# Autodesk Inventor assembly: 胴体_1
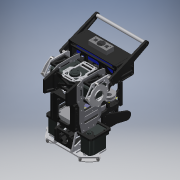
[picture p0: Inventor's stored thumbnail of the model, 180x180]
Saved by Autodesk Inventor 2018 (Build 220112000, 112)
## iProperties
Created: 2016-05-03
Part Number: 胴体_1
Document SubType Name: Assembly
Designer: hiroaki
Mass: 1394.39 g
Surface Area: 4542.63 cm^2
Volume: 847.153 cm^3
Density: 1.64598 g/cm^3
Author: hiroaki
## Documents named in this file (26)
- C:\Users\taka\Documents\github\OpenPlatform\mechanism\OpenPlatform_ver3_0\上半身\胴体\胴体_1.iam
- C:\Users\taka\Documents\github\OpenPlatform\mechanism\OpenPlatform_ver3_0\既製品\B3M11xx.ipt
- C:\Users\taka\Documents\github\OpenPlatform\mechanism\OpenPlatform_ver3_0\既製品\B3M10xx.ipt
- C:\Users\taka\Documents\github\OpenPlatform\mechanism\OpenPlatform_ver3_0\上半身\胴体\胴体_メインフレーム_1_1.ipt
- C:\Users\taka\Documents\github\OpenPlatform\mechanism\OpenPlatform_ver3_0\下半身\付け根ロール\付け根ロール_サブフレーム_1_3.ipt
- C:\Users\taka\Documents\github\OpenPlatform\mechanism\OpenPlatform_ver3_0\上半身\胴体\胴体_メインフレーム_1_2.ipt
- C:\Users\taka\Documents\github\OpenPlatform\mechanism\OpenPlatform_ver3_0\上半身\胴体\胴体_サブフレーム_1_1.ipt
- C:\Users\taka\Documents\github\OpenPlatform\mechanism\OpenPlatform_ver3_0\上半身\胴体\胴体_サブフレーム_1_2.ipt
- C:\Users\taka\Documents\github\OpenPlatform\mechanism\OpenPlatform_ver3_0\上半身\胴体\胴体_サブフレーム_1_3.ipt
- C:\Users\taka\Documents\github\OpenPlatform\mechanism\OpenPlatform_ver3_0\上半身\胴体\胴体_サブフレーム_1_4.ipt
- C:\Users\taka\Documents\github\OpenPlatform\mechanism\OpenPlatform_ver3_0\上半身\胴体\胴体_サブフレーム_1_6.ipt
- C:\Users\taka\Documents\github\OpenPlatform\mechanism\OpenPlatform_ver3_0\上半身\胴体\胴体_サブフレーム_1_6_MIR.ipt
- C:\Users\taka\Documents\github\OpenPlatform\mechanism\OpenPlatform_ver3_0\上半身\胴体\胴体_サブフレーム_1_1_MIR.ipt
- C:\Users\taka\Documents\github\OpenPlatform\mechanism\OpenPlatform_ver3_0\上半身\胴体\胴体_サブフレーム_1_7.ipt
- C:\Users\taka\Documents\github\OpenPlatform\mechanism\OpenPlatform_ver3_0\上半身\胴体\胴体_サブフレーム_1_7_MIR.ipt
- C:\Users\taka\Documents\github\OpenPlatform\mechanism\OpenPlatform_ver3_0\上半身\胴体\胴体_サブフレーム_1_9.ipt
- C:\Users\taka\Documents\github\OpenPlatform\mechanism\OpenPlatform_ver3_0\上半身\胴体\胴体_メインフレーム_1_12.ipt
- C:\Users\taka\Documents\github\OpenPlatform\mechanism\OpenPlatform_ver3_0\上半身\胴体\胴体_メインフレーム_1_13.ipt
- C:\Users\taka\Documents\github\OpenPlatform\mechanism\OpenPlatform_ver3_0\上半身\胴体\胴体_サブフレーム_1_10.ipt
- C:\Users\taka\Documents\github\OpenPlatform\mechanism\OpenPlatform_ver3_0\上半身\胴体\胴体_サブフレーム_1_11.ipt
- C:\Users\taka\Documents\github\OpenPlatform\mechanism\OpenPlatform_ver3_0\既製品\SLCG5_5-6.ipt
- C:\Users\taka\Documents\github\OpenPlatform\mechanism\OpenPlatform_ver3_0\既製品\ALSFB6-66.ipt
- C:\Users\taka\Documents\github\OpenPlatform\mechanism\OpenPlatform_ver3_0\上半身\コックピット\コックピット_2\コックピット_2.iam
- C:\Users\taka\Documents\github\OpenPlatform\mechanism\OpenPlatform_ver3_0\上半身\胴体\胴体_サブフレーム_1_12.ipt
- C:\Users\taka\Documents\github\OpenPlatform\mechanism\OpenPlatform_ver3_0\既製品\AETTF8-135-M3-N3.ipt
- C:\Users\taka\Documents\github\OpenPlatform\mechanism\OpenPlatform_ver3_0\既製品\SLCG5_5-8.ipt
## Components (60 placed, 24 different names)
1. 胴体_メインフレーム_1_1:1 — 挿入:1, 挿入:2, 挿入:3, 挿入:4, 挿入:5, 挿入:6, 挿入:43, 挿入:44, 挿入:120, 挿入:121, 挿入:194, 挿入:195, 挿入:196, 挿入:197, 挿入:198, 挿入:199, 挿入:200, 挿入:201, 角度:44
2. 付け根ロール_サブフレーム_1_3:1 — 挿入:218, 挿入:219, 挿入:220, 挿入:221
3. 胴体_メインフレーム_1_2:1 — 挿入:23, 挿入:24, 挿入:25, 挿入:28
4. 胴体_メインフレーム_1_12:1 — 挿入:148, 挿入:149, 挿入:150, 挿入:151
5. 胴体_サブフレーム_1_1:1 — 挿入:43, 挿入:44, 挿入:118, 挿入:119, メイト:9, メイト:10, メイト:11
6. 胴体_サブフレーム_1_2:1 — フラッシュ:1, メイト:3, メイト:4
7. 胴体_サブフレーム_1_3:1 — 挿入:150, 挿入:151, 挿入:162, 挿入:163, 挿入:168, 挿入:169, 挿入:192, 挿入:193, 挿入:228, 挿入:229, メイト:4, 挿入:231, 挿入:232, 挿入:236
8. 胴体_サブフレーム_1_4:1 — 挿入:57, 挿入:58, 挿入:148, 挿入:149, 挿入:152, 挿入:153, 挿入:206, 挿入:207, 挿入:208, 挿入:209, 挿入:248, 挿入:249
9. 胴体_サブフレーム_1_6:1 — 挿入:118, 挿入:119
10. 胴体_サブフレーム_1_7:1 — 挿入:231, 挿入:232
11. 胴体_サブフレーム_1_9:1 — 挿入:133, 挿入:134, 挿入:135
12. 胴体_サブフレーム_1_10:1 — 挿入:173, 挿入:174, 挿入:175, 挿入:176, 挿入:179, 挿入:188, 挿入:189
13. 胴体_サブフレーム_1_11:1 — 挿入:182, 挿入:183, 挿入:184, 挿入:185, 挿入:186, 挿入:187
14. 胴体_サブフレーム_1_12:1 — 挿入:247, 角度:35, 角度:36, 挿入:250, 挿入:251
15. 胴体_メインフレーム_1_13:1 — 挿入:188, 挿入:189, 挿入:190, 挿入:191, 挿入:192, 挿入:193
16. B3M11xx:5 — 挿入:175, 挿入:176, 挿入:179, 挿入:182, 挿入:183, 挿入:185, 挿入:186
17. B3M11xx:4 — 挿入:57, 挿入:58, 挿入:133, 挿入:134, 挿入:135, 角度:31, 角度:39
18. B3M11xx:3 — 角度:1, 挿入:76, 挿入:77, 挿入:130, 挿入:131, 挿入:132
19. B3M11xx:2 — 挿入:2, 挿入:4, 挿入:5, 挿入:23, 挿入:25, 角度:23, 角度:43
20. B3M11xx:1 — 角度:1, 挿入:1, 挿入:3, 挿入:6, 挿入:24, 挿入:28
21. SLCG5_5-6:1 — 挿入:200, 挿入:218, 角度:27, 角度:29
22. SLCG5_5-6:2 — 挿入:196, 挿入:222, 角度:25, 角度:28, 角度:43
23. SLCG5_5-6:3 — 挿入:198, 挿入:220, 角度:29
24. SLCG5_5-6:4 — 挿入:199, 挿入:219, 角度:30
25. SLCG5_5-6:5 — 挿入:204, 挿入:217, 角度:34
26. SLCG5_5-6:6 — 挿入:202, 挿入:216, 角度:42
27. SLCG5_5-6:7 — 挿入:197, 挿入:225, 角度:26
28. SLCG5_5-6:8 — 挿入:201, 挿入:221, 角度:28, 角度:30
29. SLCG5_5-6:9 — 挿入:206, 挿入:212, 角度:40
30. SLCG5_5-6:10 — 挿入:205, 挿入:215, 角度:41
31. SLCG5_5-6:11 — 挿入:203, 挿入:214, 角度:33, 角度:34
32. SLCG5_5-6:12 — 挿入:195, 挿入:224, 角度:25
33. SLCG5_5-6:13 — 挿入:207, 挿入:213, 角度:32
34. SLCG5_5-6:14 — 挿入:208, 挿入:211, 角度:31, 角度:32, 角度:33
35. SLCG5_5-6:15 — 挿入:209, 挿入:210, 角度:39, 角度:40, 角度:41, 角度:42
36. SLCG5_5-6:16 — 挿入:194, 挿入:223, 角度:23, 角度:26, 角度:27
37. ALSFB6-66:1 — 挿入:229, 挿入:230, メイト:3, メイト:9
38. ALSFB6-66:2 — 挿入:227, 挿入:228, メイト:1, メイト:2
39. ALSFB6-66:3 — メイト:10, メイト:11, 挿入:235, 挿入:236
40. コックピット_2:1 [sub-assembly] — 角度:44, メイト:14, メイト:15
41. AETTF8-135-M3-N3:1 — 挿入:246, 挿入:247
42. SLCG5_5-8:1 — 角度:38, 挿入:252, メイト:12
43. SLCG5_5-8:2 — 挿入:249, 角度:35, 挿入:251
44. SLCG5_5-8:3 — 角度:37, 挿入:253, メイト:13
45. SLCG5_5-8:4 — 挿入:248, 角度:36, 挿入:250
46. 胴体_サブフレーム_1_12:2 — 挿入:246, 角度:37, 角度:38, 挿入:252, 挿入:253
47. 胴体_メインフレーム_1_13:2 — 挿入:168, 挿入:169, 挿入:170, 挿入:171, 挿入:173, 挿入:174, 挿入:184, 挿入:187
48. 胴体_メインフレーム_1_12:2 — 挿入:152, 挿入:153, 挿入:162, 挿入:163
49. 胴体_メインフレーム_1_12:3 — 挿入:154, 挿入:155, 挿入:156, 挿入:157
50. 胴体_メインフレーム_1_12:4 — 挿入:158, 挿入:159, 挿入:160, 挿入:161
51. 胴体_サブフレーム_1_9:2 — 挿入:130, 挿入:131, 挿入:132
52. 胴体_サブフレーム_1_7_MIR:1 — 挿入:233, 挿入:234
53. 胴体_サブフレーム_1_6_MIR:1 — 挿入:122, 挿入:123
54. 付け根ロール_サブフレーム_1_3:2 — 挿入:222, 挿入:223, 挿入:224, 挿入:225
55. 付け根ロール_サブフレーム_1_3:3 — 挿入:210, 挿入:211, 挿入:212, 挿入:213
56. 付け根ロール_サブフレーム_1_3:4 — 挿入:214, 挿入:215, 挿入:216, 挿入:217
57. 胴体_サブフレーム_1_1_MIR:1 — 挿入:120, 挿入:121, 挿入:122, 挿入:123, メイト:7
58. 胴体_サブフレーム_1_2:2 — メイト:1, フラッシュ:1, メイト:2, メイト:5, メイト:7
59. 胴体_サブフレーム_1_3:2 — 挿入:156, 挿入:157, 挿入:160, 挿入:161, 挿入:170, 挿入:171, 挿入:190, 挿入:191, 挿入:227, 挿入:230, メイト:5, 挿入:233, 挿入:234, 挿入:235, メイト:14, メイト:15
60. 胴体_サブフレーム_1_4:2 — 挿入:76, 挿入:77, 挿入:154, 挿入:155, 挿入:158, 挿入:159, 挿入:202, 挿入:203, 挿入:204, 挿入:205, メイト:12, メイト:13
## Relationships (151: Insert 115, Angle 22, Mate 13, Flush 1)
- 角度:1 [Angle] (0 deg): B3M11xx:3 ↔ B3M11xx:1
- 挿入:1 [Insert]: 胴体_メインフレーム_1_1:1 ↔ B3M11xx:1
- 挿入:2 [Insert]: 胴体_メインフレーム_1_1:1 ↔ B3M11xx:2
- 挿入:3 [Insert]: 胴体_メインフレーム_1_1:1 ↔ B3M11xx:1
- 挿入:4 [Insert]: 胴体_メインフレーム_1_1:1 ↔ B3M11xx:2
- 挿入:5 [Insert]: 胴体_メインフレーム_1_1:1 ↔ B3M11xx:2
- 挿入:6 [Insert]: 胴体_メインフレーム_1_1:1 ↔ B3M11xx:1
- 挿入:23 [Insert]: 胴体_メインフレーム_1_2:1 ↔ B3M11xx:2
- 挿入:24 [Insert]: 胴体_メインフレーム_1_2:1 ↔ B3M11xx:1
- 挿入:25 [Insert]: 胴体_メインフレーム_1_2:1 ↔ B3M11xx:2
- 挿入:28 [Insert]: 胴体_メインフレーム_1_2:1 ↔ B3M11xx:1
- 挿入:43 [Insert]: 胴体_メインフレーム_1_1:1 ↔ 胴体_サブフレーム_1_1:1
- 挿入:44 [Insert]: 胴体_メインフレーム_1_1:1 ↔ 胴体_サブフレーム_1_1:1
- 挿入:57 [Insert]: 胴体_サブフレーム_1_4:1 ↔ B3M11xx:4
- 挿入:58 [Insert]: 胴体_サブフレーム_1_4:1 ↔ B3M11xx:4
- 挿入:76 [Insert]: B3M11xx:3 ↔ 胴体_サブフレーム_1_4:2
- 挿入:77 [Insert]: B3M11xx:3 ↔ 胴体_サブフレーム_1_4:2
- 挿入:118 [Insert]: 胴体_サブフレーム_1_1:1 ↔ 胴体_サブフレーム_1_6:1
- 挿入:119 [Insert]: 胴体_サブフレーム_1_1:1 ↔ 胴体_サブフレーム_1_6:1
- 挿入:120 [Insert]: 胴体_メインフレーム_1_1:1 ↔ 胴体_サブフレーム_1_1_MIR:1
- 挿入:121 [Insert]: 胴体_メインフレーム_1_1:1 ↔ 胴体_サブフレーム_1_1_MIR:1
- 挿入:122 [Insert]: 胴体_サブフレーム_1_6_MIR:1 ↔ 胴体_サブフレーム_1_1_MIR:1
- 挿入:123 [Insert]: 胴体_サブフレーム_1_6_MIR:1 ↔ 胴体_サブフレーム_1_1_MIR:1
- 挿入:130 [Insert]: B3M11xx:3 ↔ 胴体_サブフレーム_1_9:2
- 挿入:131 [Insert]: B3M11xx:3 ↔ 胴体_サブフレーム_1_9:2
- 挿入:132 [Insert]: B3M11xx:3 ↔ 胴体_サブフレーム_1_9:2
- 挿入:133 [Insert]: 胴体_サブフレーム_1_9:1 ↔ B3M11xx:4
- 挿入:134 [Insert]: 胴体_サブフレーム_1_9:1 ↔ B3M11xx:4
- 挿入:135 [Insert]: 胴体_サブフレーム_1_9:1 ↔ B3M11xx:4
- 挿入:148 [Insert]: 胴体_メインフレーム_1_12:1 ↔ 胴体_サブフレーム_1_4:1
- 挿入:149 [Insert]: 胴体_メインフレーム_1_12:1 ↔ 胴体_サブフレーム_1_4:1
- 挿入:150 [Insert]: 胴体_メインフレーム_1_12:1 ↔ 胴体_サブフレーム_1_3:1
- 挿入:151 [Insert]: 胴体_メインフレーム_1_12:1 ↔ 胴体_サブフレーム_1_3:1
- 挿入:152 [Insert]: 胴体_サブフレーム_1_4:1 ↔ 胴体_メインフレーム_1_12:2
- 挿入:153 [Insert]: 胴体_サブフレーム_1_4:1 ↔ 胴体_メインフレーム_1_12:2
- 挿入:154 [Insert]: 胴体_メインフレーム_1_12:3 ↔ 胴体_サブフレーム_1_4:2
- 挿入:155 [Insert]: 胴体_メインフレーム_1_12:3 ↔ 胴体_サブフレーム_1_4:2
- 挿入:156 [Insert]: 胴体_メインフレーム_1_12:3 ↔ 胴体_サブフレーム_1_3:2
- 挿入:157 [Insert]: 胴体_メインフレーム_1_12:3 ↔ 胴体_サブフレーム_1_3:2
- 挿入:158 [Insert]: 胴体_メインフレーム_1_12:4 ↔ 胴体_サブフレーム_1_4:2
- 挿入:159 [Insert]: 胴体_メインフレーム_1_12:4 ↔ 胴体_サブフレーム_1_4:2
- 挿入:160 [Insert]: 胴体_メインフレーム_1_12:4 ↔ 胴体_サブフレーム_1_3:2
- 挿入:161 [Insert]: 胴体_メインフレーム_1_12:4 ↔ 胴体_サブフレーム_1_3:2
- 挿入:162 [Insert]: 胴体_サブフレーム_1_3:1 ↔ 胴体_メインフレーム_1_12:2
- 挿入:163 [Insert]: 胴体_サブフレーム_1_3:1 ↔ 胴体_メインフレーム_1_12:2
- 挿入:168 [Insert]: 胴体_サブフレーム_1_3:1 ↔ 胴体_メインフレーム_1_13:2
- 挿入:169 [Insert]: 胴体_サブフレーム_1_3:1 ↔ 胴体_メインフレーム_1_13:2
- 挿入:170 [Insert]: 胴体_メインフレーム_1_13:2 ↔ 胴体_サブフレーム_1_3:2
- 挿入:171 [Insert]: 胴体_メインフレーム_1_13:2 ↔ 胴体_サブフレーム_1_3:2
- 挿入:173 [Insert]: 胴体_サブフレーム_1_10:1 ↔ 胴体_メインフレーム_1_13:2
- 挿入:174 [Insert]: 胴体_サブフレーム_1_10:1 ↔ 胴体_メインフレーム_1_13:2
- 挿入:175 [Insert]: 胴体_サブフレーム_1_10:1 ↔ B3M11xx:5
- 挿入:176 [Insert]: 胴体_サブフレーム_1_10:1 ↔ B3M11xx:5
- 挿入:179 [Insert]: 胴体_サブフレーム_1_10:1 ↔ B3M11xx:5
- 挿入:182 [Insert]: 胴体_サブフレーム_1_11:1 ↔ B3M11xx:5
- 挿入:183 [Insert]: 胴体_サブフレーム_1_11:1 ↔ B3M11xx:5
- 挿入:184 [Insert]: 胴体_サブフレーム_1_11:1 ↔ 胴体_メインフレーム_1_13:2
- 挿入:185 [Insert]: 胴体_サブフレーム_1_11:1 ↔ B3M11xx:5
- 挿入:186 [Insert]: 胴体_サブフレーム_1_11:1 ↔ B3M11xx:5
- 挿入:187 [Insert]: 胴体_サブフレーム_1_11:1 ↔ 胴体_メインフレーム_1_13:2
- 挿入:188 [Insert]: 胴体_サブフレーム_1_10:1 ↔ 胴体_メインフレーム_1_13:1
- 挿入:189 [Insert]: 胴体_サブフレーム_1_10:1 ↔ 胴体_メインフレーム_1_13:1
- 挿入:190 [Insert]: 胴体_メインフレーム_1_13:1 ↔ 胴体_サブフレーム_1_3:2
- 挿入:191 [Insert]: 胴体_メインフレーム_1_13:1 ↔ 胴体_サブフレーム_1_3:2
- 挿入:192 [Insert]: 胴体_サブフレーム_1_3:1 ↔ 胴体_メインフレーム_1_13:1
- 挿入:193 [Insert]: 胴体_サブフレーム_1_3:1 ↔ 胴体_メインフレーム_1_13:1
- 挿入:194 [Insert]: 胴体_メインフレーム_1_1:1 ↔ SLCG5_5-6:16
- 挿入:195 [Insert]: 胴体_メインフレーム_1_1:1 ↔ SLCG5_5-6:12
- 挿入:196 [Insert]: 胴体_メインフレーム_1_1:1 ↔ SLCG5_5-6:2
- 挿入:197 [Insert]: 胴体_メインフレーム_1_1:1 ↔ SLCG5_5-6:7
- 挿入:198 [Insert]: 胴体_メインフレーム_1_1:1 ↔ SLCG5_5-6:3
- 挿入:199 [Insert]: 胴体_メインフレーム_1_1:1 ↔ SLCG5_5-6:4
- 挿入:200 [Insert]: 胴体_メインフレーム_1_1:1 ↔ SLCG5_5-6:1
- 挿入:201 [Insert]: 胴体_メインフレーム_1_1:1 ↔ SLCG5_5-6:8
- 挿入:202 [Insert]: SLCG5_5-6:6 ↔ 胴体_サブフレーム_1_4:2
- 挿入:203 [Insert]: SLCG5_5-6:11 ↔ 胴体_サブフレーム_1_4:2
- 挿入:204 [Insert]: SLCG5_5-6:5 ↔ 胴体_サブフレーム_1_4:2
- 挿入:205 [Insert]: SLCG5_5-6:10 ↔ 胴体_サブフレーム_1_4:2
- 挿入:206 [Insert]: 胴体_サブフレーム_1_4:1 ↔ SLCG5_5-6:9
- 挿入:207 [Insert]: 胴体_サブフレーム_1_4:1 ↔ SLCG5_5-6:13
- 挿入:208 [Insert]: 胴体_サブフレーム_1_4:1 ↔ SLCG5_5-6:14
- 挿入:209 [Insert]: 胴体_サブフレーム_1_4:1 ↔ SLCG5_5-6:15
- 挿入:210 [Insert]: SLCG5_5-6:15 ↔ 付け根ロール_サブフレーム_1_3:3
- 挿入:211 [Insert]: SLCG5_5-6:14 ↔ 付け根ロール_サブフレーム_1_3:3
- 挿入:212 [Insert]: SLCG5_5-6:9 ↔ 付け根ロール_サブフレーム_1_3:3
- 挿入:213 [Insert]: SLCG5_5-6:13 ↔ 付け根ロール_サブフレーム_1_3:3
- 挿入:214 [Insert]: SLCG5_5-6:11 ↔ 付け根ロール_サブフレーム_1_3:4
- 挿入:215 [Insert]: SLCG5_5-6:10 ↔ 付け根ロール_サブフレーム_1_3:4
- 挿入:216 [Insert]: SLCG5_5-6:6 ↔ 付け根ロール_サブフレーム_1_3:4
- 挿入:217 [Insert]: SLCG5_5-6:5 ↔ 付け根ロール_サブフレーム_1_3:4
- 挿入:218 [Insert]: 付け根ロール_サブフレーム_1_3:1 ↔ SLCG5_5-6:1
- 挿入:219 [Insert]: 付け根ロール_サブフレーム_1_3:1 ↔ SLCG5_5-6:4
- 挿入:220 [Insert]: 付け根ロール_サブフレーム_1_3:1 ↔ SLCG5_5-6:3
- 挿入:221 [Insert]: 付け根ロール_サブフレーム_1_3:1 ↔ SLCG5_5-6:8
- 挿入:222 [Insert]: SLCG5_5-6:2 ↔ 付け根ロール_サブフレーム_1_3:2
- 挿入:223 [Insert]: SLCG5_5-6:16 ↔ 付け根ロール_サブフレーム_1_3:2
- 挿入:224 [Insert]: SLCG5_5-6:12 ↔ 付け根ロール_サブフレーム_1_3:2
- 挿入:225 [Insert]: SLCG5_5-6:7 ↔ 付け根ロール_サブフレーム_1_3:2
- 角度:23 [Angle] (0 deg): B3M11xx:2 ↔ SLCG5_5-6:16
- 角度:25 [Angle] (0 deg): SLCG5_5-6:2 ↔ SLCG5_5-6:12
- 角度:26 [Angle] (0 deg): SLCG5_5-6:7 ↔ SLCG5_5-6:16
- 角度:27 [Angle] (0 deg): SLCG5_5-6:1 ↔ SLCG5_5-6:16
- 角度:28 [Angle] (0 deg): SLCG5_5-6:2 ↔ SLCG5_5-6:8
- 角度:29 [Angle] (0 deg): SLCG5_5-6:1 ↔ SLCG5_5-6:3
- 角度:30 [Angle] (0 deg): SLCG5_5-6:4 ↔ SLCG5_5-6:8
- 角度:31 [Angle] (0 deg): B3M11xx:4 ↔ SLCG5_5-6:14
- 角度:32 [Angle] (0 deg): SLCG5_5-6:13 ↔ SLCG5_5-6:14
- 角度:33 [Angle] (0 deg): SLCG5_5-6:11 ↔ SLCG5_5-6:14
- 角度:34 [Angle] (0 deg): SLCG5_5-6:5 ↔ SLCG5_5-6:11
- 挿入:227 [Insert]: ALSFB6-66:2 ↔ 胴体_サブフレーム_1_3:2
- 挿入:228 [Insert]: 胴体_サブフレーム_1_3:1 ↔ ALSFB6-66:2
- 挿入:229 [Insert]: 胴体_サブフレーム_1_3:1 ↔ ALSFB6-66:1
- 挿入:230 [Insert]: ALSFB6-66:1 ↔ 胴体_サブフレーム_1_3:2
- メイト:1 [Mate] (0.005 mm): ALSFB6-66:2 ↔ 胴体_サブフレーム_1_2:2
- フラッシュ:1 [Flush]: 胴体_サブフレーム_1_2:1 ↔ 胴体_サブフレーム_1_2:2
- メイト:2 [Mate] (0.05 mm): ALSFB6-66:2 ↔ 胴体_サブフレーム_1_2:2
- メイト:3 [Mate] (0.005 mm): 胴体_サブフレーム_1_2:1 ↔ ALSFB6-66:1
- メイト:4 [Mate]: 胴体_サブフレーム_1_2:1 ↔ 胴体_サブフレーム_1_3:1
- メイト:5 [Mate]: 胴体_サブフレーム_1_2:2 ↔ 胴体_サブフレーム_1_3:2
- メイト:7 [Mate]: 胴体_サブフレーム_1_1_MIR:1 ↔ 胴体_サブフレーム_1_2:2
- 挿入:231 [Insert]: 胴体_サブフレーム_1_3:1 ↔ 胴体_サブフレーム_1_7:1
- 挿入:232 [Insert]: 胴体_サブフレーム_1_3:1 ↔ 胴体_サブフレーム_1_7:1
- 挿入:233 [Insert]: 胴体_サブフレーム_1_7_MIR:1 ↔ 胴体_サブフレーム_1_3:2
- 挿入:234 [Insert]: 胴体_サブフレーム_1_7_MIR:1 ↔ 胴体_サブフレーム_1_3:2
- メイト:9 [Mate] (0.005 mm): 胴体_サブフレーム_1_1:1 ↔ ALSFB6-66:1
- メイト:10 [Mate] (0.005 mm): 胴体_サブフレーム_1_1:1 ↔ ALSFB6-66:3
- メイト:11 [Mate] (0.005 mm): 胴体_サブフレーム_1_1:1 ↔ ALSFB6-66:3
- 挿入:235 [Insert]: ALSFB6-66:3 ↔ 胴体_サブフレーム_1_3:2
- 挿入:236 [Insert]: 胴体_サブフレーム_1_3:1 ↔ ALSFB6-66:3
- 挿入:246 [Insert]: AETTF8-135-M3-N3:1 ↔ 胴体_サブフレーム_1_12:2
- 挿入:247 [Insert]: 胴体_サブフレーム_1_12:1 ↔ AETTF8-135-M3-N3:1
- 挿入:248 [Insert]: 胴体_サブフレーム_1_4:1 ↔ SLCG5_5-8:4
- 挿入:249 [Insert]: 胴体_サブフレーム_1_4:1 ↔ SLCG5_5-8:2
- 角度:35 [Angle] (0 deg): 胴体_サブフレーム_1_12:1 ↔ SLCG5_5-8:2
- 角度:36 [Angle] (0 deg): 胴体_サブフレーム_1_12:1 ↔ SLCG5_5-8:4
- 挿入:250 [Insert]: 胴体_サブフレーム_1_12:1 ↔ SLCG5_5-8:4
- 挿入:251 [Insert]: 胴体_サブフレーム_1_12:1 ↔ SLCG5_5-8:2
- 角度:37 [Angle] (0 deg): SLCG5_5-8:3 ↔ 胴体_サブフレーム_1_12:2
- 角度:38 [Angle] (0 deg): SLCG5_5-8:1 ↔ 胴体_サブフレーム_1_12:2
- 挿入:252 [Insert]: SLCG5_5-8:1 ↔ 胴体_サブフレーム_1_12:2
- 挿入:253 [Insert]: SLCG5_5-8:3 ↔ 胴体_サブフレーム_1_12:2
- メイト:12 [Mate]: SLCG5_5-8:1 ↔ 胴体_サブフレーム_1_4:2
- メイト:13 [Mate]: SLCG5_5-8:3 ↔ 胴体_サブフレーム_1_4:2
- 角度:39 [Angle] (0 deg): B3M11xx:4 ↔ SLCG5_5-6:15
- 角度:40 [Angle] (0 deg): SLCG5_5-6:9 ↔ SLCG5_5-6:15
- 角度:41 [Angle] (0 deg): SLCG5_5-6:10 ↔ SLCG5_5-6:15
- 角度:42 [Angle] (0 deg): SLCG5_5-6:6 ↔ SLCG5_5-6:15
- 角度:43 [Angle] (0 deg): B3M11xx:2 ↔ SLCG5_5-6:2
- 角度:44 [Angle] (180 deg): 胴体_メインフレーム_1_1:1 ↔ コックピット_2:1
- メイト:14 [Mate]: コックピット_2:1 ↔ 胴体_サブフレーム_1_3:2
- メイト:15 [Mate]: コックピット_2:1 ↔ 胴体_サブフレーム_1_3:2
